# Autodesk Inventor assembly: Bein
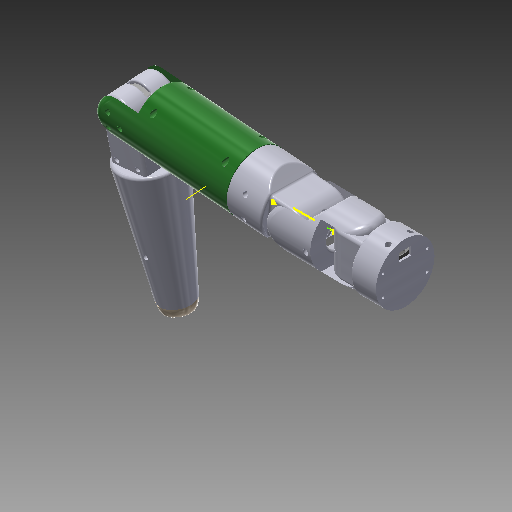
[picture p0: Inventor's stored thumbnail of the model, 512x512]
Saved by Autodesk Inventor 2018 (Build 220112000, 112)
## iProperties
Part Number: Bein
Material: Generisch
Document SubType Name: Assembly
Designer: Jochen Alt
Mass: 312.865 g
Surface Area: 2260 cm^2
Volume: 258.484 cm^3
Density: 1.21038 g/cm^3
Author: Jochen Alt
## Documents named in this file (10)
- D:\Projects\Manfred\cad\Inventor\Leg.iam
- D:\Projects\Manfred\cad\Inventor\HipJoint.ipt
- D:\Projects\Manfred\cad\Inventor\Hip.ipt
- D:\Projects\Manfred\cad\Inventor\Foot.ipt
- D:\Projects\Manfred\cad\Inventor\Herkulex DRS-010x\HerkuleX DRS-0101.iam
- D:\Projects\Manfred\cad\Inventor\Rillenkugellager 11x7x3 inafag smr117.ipt
- D:\Projects\Manfred\cad\Inventor\Servobackaxis.ipt
- D:\Projects\Manfred\cad\Inventor\Thigh.iam
- D:\Projects\Manfred\cad\Inventor\abstandsbolzen M2 10mm.ipt
- D:\Projects\Manfred\cad\Inventor\VL6180X\VL6180X-Time_of_Flight_Sensor.ipt
## Components (13 placed, 9 different names)
1. Hip:3 — Passend:83, Winkel:1, Passend:84, Passend:154
2. HipJoint:1 — Passend:100, Passend:101, Passend:102, Passend:103, Passend:110, Passend:111, Passend:155, Passend:156
3. Foot:1 — Passend:118, Passend:119, Passend:120, Passend:144, Winkel:2, Passend:163, Passend:164, Passend:165, Passend:166, Passend:167, Passend:168
4. HerkuleX DRS-0101:1 [sub-assembly] — Passend:83, Winkel:1, Passend:84, Passend:86
5. Rillenkugellager 11x7x3 inafag smr117:1 — Passend:86, Passend:87, Passend:88, Passend:154
6. Servobackaxis:1 — Passend:87, Passend:88, Passend:155, Passend:156
7. abstandsbolzen M2 10mm:1 — Passend:101, Passend:102
8. abstandsbolzen M2 10mm:2 — Passend:100, Passend:103
9. Thigh:1 [sub-assembly] — Passend:110, Passend:111, Passend:144, Passend:147
10. HerkuleX DRS-0101:2 [sub-assembly] — Passend:118, Passend:119, Passend:146, Winkel:2
11. Servobackaxis:2 — Passend:122, Passend:145, Passend:147
12. Rillenkugellager 11x7x3 inafag smr117:2 — Passend:120, Passend:122, Passend:145, Passend:146
13. VL6180X-Time_of_Flight_Sensor:1 — Passend:163, Passend:164, Passend:165, Passend:166, Passend:167, Passend:168
## Relationships (30: Mate 28, Angle 2)
- Passend:83 [Mate]: Hip:3 ↔ HerkuleX DRS-0101:1
- Winkel:1 [Angle] (90 deg): Hip:3 ↔ HerkuleX DRS-0101:1
- Passend:84 [Mate] (0.1 mm): Hip:3 ↔ HerkuleX DRS-0101:1
- Passend:86 [Mate] (0.5 mm): HerkuleX DRS-0101:1 ↔ Rillenkugellager 11x7x3 inafag smr117:1
- Passend:87 [Mate]: Rillenkugellager 11x7x3 inafag smr117:1 ↔ Servobackaxis:1
- Passend:88 [Mate] (0.1 mm): Rillenkugellager 11x7x3 inafag smr117:1 ↔ Servobackaxis:1
- Passend:100 [Mate]: HipJoint:1 ↔ abstandsbolzen M2 10mm:2
- Passend:101 [Mate]: HipJoint:1 ↔ abstandsbolzen M2 10mm:1
- Passend:102 [Mate] (1 mm): HipJoint:1 ↔ abstandsbolzen M2 10mm:1
- Passend:103 [Mate] (1 mm): HipJoint:1 ↔ abstandsbolzen M2 10mm:2
- Passend:110 [Mate]: HipJoint:1 ↔ Thigh:1
- Passend:111 [Mate] (0.1 mm): HipJoint:1 ↔ Thigh:1
- Passend:118 [Mate]: Foot:1 ↔ HerkuleX DRS-0101:2
- Passend:119 [Mate] (0.1 mm): Foot:1 ↔ HerkuleX DRS-0101:2
- Passend:120 [Mate]: Foot:1 ↔ Rillenkugellager 11x7x3 inafag smr117:2
- Passend:122 [Mate]: Servobackaxis:2 ↔ Rillenkugellager 11x7x3 inafag smr117:2
- Passend:144 [Mate]: Foot:1 ↔ Thigh:1
- Passend:145 [Mate]: Servobackaxis:2 ↔ Rillenkugellager 11x7x3 inafag smr117:2
- Passend:146 [Mate] (0.5 mm): HerkuleX DRS-0101:2 ↔ Rillenkugellager 11x7x3 inafag smr117:2
- Passend:147 [Mate]: Thigh:1 ↔ Servobackaxis:2
- Passend:154 [Mate]: Hip:3 ↔ Rillenkugellager 11x7x3 inafag smr117:1
- Passend:155 [Mate]: HipJoint:1 ↔ Servobackaxis:1
- Passend:156 [Mate] (0.1 mm): HipJoint:1 ↔ Servobackaxis:1
- Winkel:2 [Angle] (90 deg): Foot:1 ↔ HerkuleX DRS-0101:2
- Passend:163 [Mate]: Foot:1 ↔ VL6180X-Time_of_Flight_Sensor:1
- Passend:164 [Mate]: Foot:1 ↔ VL6180X-Time_of_Flight_Sensor:1
- Passend:165 [Mate]: Foot:1 ↔ VL6180X-Time_of_Flight_Sensor:1
- Passend:166 [Mate]: Foot:1 ↔ VL6180X-Time_of_Flight_Sensor:1
- Passend:167 [Mate]: Foot:1 ↔ VL6180X-Time_of_Flight_Sensor:1
- Passend:168 [Mate]: Foot:1 ↔ VL6180X-Time_of_Flight_Sensor:1
